# Autodesk Inventor assembly: powerButtonAssembly
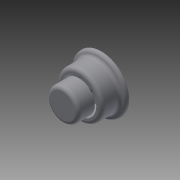
[picture p0: Inventor's stored thumbnail of the model, 180x180]
Saved by Autodesk Inventor 2014 SP2 (Build 180246200, 246)
## iProperties
Created: 2020-04-12
Part Number: powerButtonAssembly
Document SubType Name: Assembly
Designer: GauchoHP
Author: GauchoHP
## Documents named in this file (5)
- C:\Users\GauchoHP\Desktop\old_desktop\tosaerba\LAWNMOWER-ROBOT-from-Hoverboard-\LawnmowerMechanicalProject\3D PROJECT - INVENTOR 2014\power button\powerButtonAssembly.iam
- C:\Users\GauchoHP\Desktop\old_desktop\tosaerba\LAWNMOWER-ROBOT-from-Hoverboard-\LawnmowerMechanicalProject\3D PROJECT - INVENTOR 2014\power button\powerButtonPart1.ipt
- C:\Users\GauchoHP\Desktop\old_desktop\tosaerba\LAWNMOWER-ROBOT-from-Hoverboard-\LawnmowerMechanicalProject\3D PROJECT - INVENTOR 2014\power button\powerButtonPart2.ipt
- C:\Users\GauchoHP\Documents\Inventor\Content Center Files\R2014\en-US\ANSI B18.6.3(11)\ANSI B18.6.3 - 3-56 UNF - 1(10).ipt
- C:\Users\GauchoHP\Desktop\old_desktop\tosaerba\LAWNMOWER-ROBOT-from-Hoverboard-\LawnmowerMechanicalProject\3D PROJECT - INVENTOR 2014\power button\gum.ipt
## Components (4 placed, 4 different names)
1. powerButtonPart1:1 — Mate:1, Mate:2, Mate:3, Mate:4
2. powerButtonPart2:1 — Mate:1, Mate:2
3. Cross Recessed Fillister Head Machine Screw - Type II - Inch No. 3 - 56 - 1:1 — Mate:3, Mate:4, Mate:5, Mate:6
4. gum:1 — Mate:5, Mate:6
## Relationships (6: Mate 6)
- Mate:1 (10 mm): powerButtonPart1:1 ↔ powerButtonPart2:1
- Mate:2: powerButtonPart1:1 ↔ powerButtonPart2:1
- Mate:3: powerButtonPart1:1 ↔ Cross Recessed Fillister Head Machine Screw - Type II - Inch No. 3 - 56 - 1:1
- Mate:4 (1 mm): powerButtonPart1:1 ↔ Cross Recessed Fillister Head Machine Screw - Type II - Inch No. 3 - 56 - 1:1
- Mate:5: Cross Recessed Fillister Head Machine Screw - Type II - Inch No. 3 - 56 - 1:1 ↔ gum:1
- Mate:6: Cross Recessed Fillister Head Machine Screw - Type II - Inch No. 3 - 56 - 1:1 ↔ gum:1
